# Autodesk Inventor assembly: Сборка3
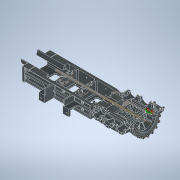
[picture p0: Inventor's stored thumbnail of the model, 180x180]
Saved by Autodesk Inventor 2021 (Build 250183000, 183)
## iProperties
Created: 2020-11-22
Part Number: Сборка3
Document SubType Name: Assembly
Designer: Тимоха
Author: Тимоха
## Documents named in this file (55)
- C:\Users\Тимоха\Desktop\КР Компрессор\compressor\Сборка3.iam
- C:\Users\Тимоха\Desktop\КР Компрессор\compressor\Верхняя часть поршня.ipt
- C:\Users\Тимоха\Desktop\КР Компрессор\compressor\Втулка.ipt
- C:\Users\Тимоха\Desktop\КР Компрессор\compressor\Гайка шток-поршень.ipt
- C:\Users\Тимоха\Desktop\КР Компрессор\compressor\Дроссельное кольцо.ipt
- C:\Users\Тимоха\Desktop\КР Компрессор\compressor\Клапан1.iam
- C:\Users\Тимоха\Desktop\КР Компрессор\compressor\Кольцо поршень-шток верх.ipt
- C:\Users\Тимоха\Desktop\КР Компрессор\compressor\Кольцо поршень-шток низ.ipt
- C:\Users\Тимоха\Desktop\КР Компрессор\compressor\Кольцо поршня.ipt
- C:\Users\Тимоха\Desktop\КР Компрессор\compressor\Кольцо сальника.ipt
- C:\Users\Тимоха\Desktop\КР Компрессор\compressor\Корпус дросселя.ipt
- C:\Users\Тимоха\Desktop\КР Компрессор\compressor\Корпус сальника.ipt
- C:\Users\Тимоха\Desktop\КР Компрессор\compressor\Крышка сальников.ipt
- C:\Users\Тимоха\Desktop\КР Компрессор\compressor\Крышка стакана.ipt
- C:\Users\Тимоха\Desktop\КР Компрессор\compressor\Крышка цилиндра 1.ipt
- C:\Users\Тимоха\Desktop\КР Компрессор\compressor\Крышка цилиндра 2.ipt
- C:\Users\Тимоха\Desktop\КР Компрессор\compressor\Нижняя часть поршня.ipt
- C:\Users\Тимоха\Desktop\КР Компрессор\compressor\Опорное кольцо.ipt
- C:\Users\Тимоха\Desktop\КР Компрессор\compressor\Прокладка клапана.ipt
- C:\Users\Тимоха\Desktop\КР Компрессор\compressor\Пружина дросселя.ipt
- C:\Users\Тимоха\Desktop\КР Компрессор\compressor\Пружина сальника.ipt
- C:\Users\Тимоха\Desktop\КР Компрессор\compressor\Стакан1.ipt
- C:\Users\Тимоха\Desktop\КР Компрессор\compressor\Цилиндр2.ipt
- C:\Users\Тимоха\Desktop\КР Компрессор\compressor\Шток.ipt
- C:\Users\Тимоха\Desktop\КР Компрессор\compressor\Прокладка сальников.ipt
- C:\Users\Тимоха\Documents\Inventor\Content Center Files\R2021\ru-RU\Stud GOST 22034-76\Шпилька M20-6g×50 ГОСТ 22034-76.ipt
- C:\Users\Тимоха\Documents\Inventor\Content Center Files\R2021\ru-RU\GOST 10450-78\Шайба 21 ГОСТ 10450-78.ipt
- C:\Users\Тимоха\Documents\Inventor\Content Center Files\R2021\ru-RU\GOST 15521-70\Гайка M20-6H ГОСТ 15521-70.ipt
- C:\Users\Тимоха\Documents\Inventor\Content Center Files\R2021\ru-RU\GOST 11371-78  A\Шайба 24 ГОСТ 11371-78.ipt
- C:\Users\Тимоха\Documents\Inventor\Content Center Files\R2021\ru-RU\Stud GOST 22038-76\Шпилька M24-6g×70 ГОСТ 22038-76.ipt
- C:\Users\Тимоха\Documents\Inventor\Content Center Files\R2021\ru-RU\Nut GOST 15524-70\Гайка M24-6H ГОСТ 15524-70.ipt
- C:\Users\Тимоха\Documents\Inventor\Content Center Files\R2021\ru-RU\Bolt GOST R 50274-92\Болт M8-6g×20-F ГОСТ Р 50274-92.ipt
- C:\Users\Тимоха\Desktop\КР Компрессор\compressor\Деталь5.ipt
- C:\Users\Тимоха\Desktop\КР Компрессор\compressor\Деталь6.ipt
- C:\Users\Тимоха\Desktop\КР Компрессор\compressor\Прокладка воды зад.ipt
- C:\Users\Тимоха\Desktop\КР Компрессор\compressor\Крышка воды зад.ipt
- C:\Users\Тимоха\Documents\Inventor\Content Center Files\R2021\ru-RU\GOST 15521-70\Гайка M10-6H ГОСТ 15521-70.ipt
- C:\Users\Тимоха\Documents\Inventor\Content Center Files\R2021\ru-RU\Stud GOST 22034-76\Шпилька M10-6g×45 ГОСТ 22034-76.ipt
- C:\Users\Тимоха\Documents\Inventor\Content Center Files\R2021\ru-RU\Washer GOST 9065-75\Шайба 12 ГОСТ 9065-75.ipt
- C:\Users\Тимоха\Desktop\КР Компрессор\compressor\Фонарь.ipt
- C:\Users\Тимоха\Documents\Inventor\Content Center Files\R2021\ru-RU\Stud GOST 22038-76\Шпилька M20-6g×80 ГОСТ 22038-76.ipt
- C:\Users\Тимоха\Documents\Inventor\Content Center Files\R2021\ru-RU\GOST 6402-70\Шайба  22 L ГОСТ 6402-70.ipt
- C:\Users\Тимоха\Documents\Inventor\Content Center Files\R2021\ru-RU\Nut GOST ISO 8673-2014\Копия Копия гайки M20x1,5-6H ГОСТ 5915-70.ipt
- C:\Users\Тимоха\Desktop\КР Компрессор\compressor\Корпус сальника перегородка 1.ipt
- C:\Users\Тимоха\Desktop\КР Компрессор\compressor\Крышка перегородки11.ipt
- C:\Users\Тимоха\Desktop\КР Компрессор\compressor\Крышка перегородки12.ipt
- C:\Users\Тимоха\Desktop\КР Компрессор\compressor\Придав перегородки1.ipt
- C:\Users\Тимоха\Desktop\КР Компрессор\compressor\Корпус маслосъемника.ipt
- C:\Users\Тимоха\Desktop\КР Компрессор\compressor\Крышка перегородки21.ipt
- C:\Users\Тимоха\Desktop\КР Компрессор\compressor\Крышка перегородки22.ipt
- C:\Users\Тимоха\Desktop\КР Компрессор\compressor\Маслосъемная пружина.ipt
- C:\Users\Тимоха\Desktop\КР Компрессор\compressor\Маслосъемное кольцо.ipt
- C:\Users\Тимоха\Documents\Inventor\Content Center Files\R2021\ru-RU\GOST 11738-84\Винт M10-6gx20 ГОСТ 11738-84.ipt
- C:\Users\Тимоха\Documents\Inventor\Content Center Files\R2021\ru-RU\GOST 11371-78  A\Шайба 12 ГОСТ 11371-78.ipt
- C:\Users\Тимоха\Documents\Inventor\Content Center Files\R2021\ru-RU\GOST 11738-84\Винт M10-6gx25 ГОСТ 11738-84.ipt
## Components (444 placed, 54 different names)
1. Верхняя часть поршня:1 — С поворотом:1, С поворотом:2, Жесткий:3, Жесткий:6
2. Втулка:1 — Жесткий:9, Жесткий:12, Жесткий:14
3. Дроссельное кольцо:1 — Жесткий:21, Жесткий:22
4. Клапан1:1 [sub-assembly] — Жесткий:11, С поворотом:4
5. Кольцо поршень-шток низ:1 — Жесткий:5
6. Кольцо поршня:1 — С поворотом:2
7. Корпус дросселя:1 — Жесткий:22, С поворотом:6, С поворотом:7
8. Крышка сальников:1 — Жесткий:72, Жесткий:73, Жесткий:143
9. Крышка стакана:1 — С поворотом:5
10. Крышка цилиндра 1:1 — Жесткий:12, С поворотом:9
11. Крышка цилиндра 2:1 — Жесткий:13, С поворотом:6, Жесткий:79, Жесткий:142, Жесткий:145, С поворотом:16
12. Нижняя часть поршня:1 — С поворотом:1, Жесткий:1, Жесткий:2, Жесткий:4, Жесткий:5
13. Опорное кольцо:1 — Жесткий:4
14. Прокладка клапана:1 — Жесткий:10, Жесткий:11
15. Пружина дросселя:1 — Жесткий:21
16. Стакан1:1 — С поворотом:4, С поворотом:5
17. Цилиндр2:1 — Жесткий:9, Жесткий:10, Жесткий:13, Жесткий:74, Жесткий:76, Жесткий:80, Заподлицо:1, Заподлицо:2, Заподлицо:5, Заподлицо:6
18. Кольцо поршня:2 — Жесткий:1, Жесткий:14
19. Кольцо поршня:3 — Жесткий:2
20. Опорное кольцо:2 — Жесткий:3
21. Гайка шток-поршень:1 — Жесткий:7, Жесткий:8
22. Кольцо поршень-шток верх:1 — Жесткий:6, Жесткий:7
23. Шток:1 — Жесткий:8
24. Прокладка сальников:1 — Жесткий:29, С поворотом:7
25. Кольцо сальника:4
26. Корпус сальника:2 — Жесткий:29, Жесткий:65
27. Пружина сальника:4
28. Кольцо сальника:5
29. Пружина сальника:5
30. Кольцо сальника:6
31. Пружина сальника:6
32. Прокладка сальников:2
33. Кольцо сальника:7
34. Корпус сальника:3 — Жесткий:69, Жесткий:73
35. Пружина сальника:7
36. Кольцо сальника:8
37. Пружина сальника:8
38. Кольцо сальника:9
39. Пружина сальника:9
40. Прокладка сальников:3
41. Кольцо сальника:10
42. Корпус сальника:4 — Жесткий:66, Жесткий:67
43. Пружина сальника:10
44. Кольцо сальника:11
45. Пружина сальника:11
46. Кольцо сальника:12
47. Пружина сальника:12
48. Прокладка сальников:4 — Жесткий:67
49. Кольцо сальника:13
50. Корпус сальника:5 — Жесткий:68
51. Пружина сальника:13
52. Кольцо сальника:14
53. Пружина сальника:14
54. Кольцо сальника:15
55. Пружина сальника:15
56. Прокладка сальников:5
57. Кольцо сальника:16
58. Корпус сальника:6 — Жесткий:68, Жесткий:69
59. Пружина сальника:16
60. Кольцо сальника:17
61. Пружина сальника:17
62. Кольцо сальника:18
63. Пружина сальника:18
64. Прокладка сальников:6
65. Кольцо сальника:19
66. Корпус сальника:7 — Жесткий:65, Жесткий:66
67. Пружина сальника:19
68. Кольцо сальника:20
69. Пружина сальника:20
70. Кольцо сальника:21
71. Пружина сальника:21
72. Кольцо сальника:22 — Жесткий:70, Жесткий:140
73. Кольцо сальника:23 — Жесткий:70, Жесткий:71, Жесткий:139
74. Кольцо сальника:24 — Жесткий:71, Жесткий:72, Жесткий:141
75. Болт ГОСТ Р 50274-92 M8-6g×20-F:2 — Жесткий:82
76. Болт ГОСТ Р 50274-92 M8-6g×20-F:3 — Жесткий:81
77. Деталь5:1 — Заподлицо:1, Заподлицо:2, Заподлицо:3, Заподлицо:4
78. Деталь6:1 — Заподлицо:3, Заподлицо:4, Жесткий:81, Жесткий:82, С поворотом:10, С поворотом:11, С поворотом:12, С поворотом:13, С поворотом:14, Жесткий:83, Жесткий:84, Жесткий:85, Жесткий:86, Жесткий:87, Жесткий:88, Жесткий:89, Жесткий:90, Жесткий:91, Жесткий:92, Жесткий:93, Жесткий:94, Жесткий:95, Жесткий:96, Жесткий:97, Жесткий:98, Жесткий:99, Жесткий:100, Жесткий:101, Жесткий:102, Жесткий:103, Жесткий:104, Жесткий:105, Жесткий:106, Жесткий:107
79. Прокладка воды зад:1 — Заподлицо:5, Заподлицо:6, Заподлицо:7, Заподлицо:8
80. Крышка воды зад:1 — Заподлицо:7, Заподлицо:8, С поворотом:15, Жесткий:108, Жесткий:109, Жесткий:110, Жесткий:111, Жесткий:112, Жесткий:113, Жесткий:114, Жесткий:115, Жесткий:116, Жесткий:117, Жесткий:118, Жесткий:119, Жесткий:120, Жесткий:121, Жесткий:122, Жесткий:123, Жесткий:124, Жесткий:125, Жесткий:126, Жесткий:127, Жесткий:128, Жесткий:129, Жесткий:130, Жесткий:131, Жесткий:132, Жесткий:133, Жесткий:134, Жесткий:135, Жесткий:136, Жесткий:137, Жесткий:138
81. Болт ГОСТ Р 50274-92 M8-6g×20-F:33 — С поворотом:14
82. Болт ГОСТ Р 50274-92 M8-6g×20-F:34 — Жесткий:85
83. Болт ГОСТ Р 50274-92 M8-6g×20-F:35 — С поворотом:11
84. Болт ГОСТ Р 50274-92 M8-6g×20-F:36 — С поворотом:10
85. Болт ГОСТ Р 50274-92 M8-6g×20-F:37 — Жесткий:83
86. Болт ГОСТ Р 50274-92 M8-6g×20-F:38 — Жесткий:84
87. Болт ГОСТ Р 50274-92 M8-6g×20-F:39 — С поворотом:12
88. Болт ГОСТ Р 50274-92 M8-6g×20-F:40 — С поворотом:13
89. Болт ГОСТ Р 50274-92 M8-6g×20-F:41 — Жесткий:91
90. Болт ГОСТ Р 50274-92 M8-6g×20-F:42 — Жесткий:90
91. Болт ГОСТ Р 50274-92 M8-6g×20-F:43 — Жесткий:87
92. Болт ГОСТ Р 50274-92 M8-6g×20-F:44 — Жесткий:86
93. Болт ГОСТ Р 50274-92 M8-6g×20-F:45 — Жесткий:89
94. Болт ГОСТ Р 50274-92 M8-6g×20-F:46 — Жесткий:93
95. Болт ГОСТ Р 50274-92 M8-6g×20-F:47 — Жесткий:88
96. Болт ГОСТ Р 50274-92 M8-6g×20-F:48 — Жесткий:92
97. Болт ГОСТ Р 50274-92 M8-6g×20-F:49 — Жесткий:99
98. Болт ГОСТ Р 50274-92 M8-6g×20-F:50 — Жесткий:98
99. Болт ГОСТ Р 50274-92 M8-6g×20-F:51 — Жесткий:97
100. Болт ГОСТ Р 50274-92 M8-6g×20-F:52 — Жесткий:94
101. Болт ГОСТ Р 50274-92 M8-6g×20-F:53 — Жесткий:95
102. Болт ГОСТ Р 50274-92 M8-6g×20-F:54 — Жесткий:102
103. Болт ГОСТ Р 50274-92 M8-6g×20-F:55 — Жесткий:100
104. Болт ГОСТ Р 50274-92 M8-6g×20-F:56 — Жесткий:101
105. Болт ГОСТ Р 50274-92 M8-6g×20-F:58 — Жесткий:106
106. Болт ГОСТ Р 50274-92 M8-6g×20-F:59 — Жесткий:104
107. Болт ГОСТ Р 50274-92 M8-6g×20-F:60 — Жесткий:96
108. Болт ГОСТ Р 50274-92 M8-6g×20-F:61 — Жесткий:107
109. Болт ГОСТ Р 50274-92 M8-6g×20-F:63 — Жесткий:103
110. Болт ГОСТ Р 50274-92 M8-6g×20-F:64 — Жесткий:105
111. Болт ГОСТ Р 50274-92 M8-6g×20-F:68 — С поворотом:15
112. Болт ГОСТ Р 50274-92 M8-6g×20-F:97 — Жесткий:108
113. Болт ГОСТ Р 50274-92 M8-6g×20-F:98 — Жесткий:110
114. Болт ГОСТ Р 50274-92 M8-6g×20-F:99 — Жесткий:109
115. Болт ГОСТ Р 50274-92 M8-6g×20-F:100 — Жесткий:111
116. Болт ГОСТ Р 50274-92 M8-6g×20-F:101 — Жесткий:113
117. Болт ГОСТ Р 50274-92 M8-6g×20-F:102 — Жесткий:112
118. Болт ГОСТ Р 50274-92 M8-6g×20-F:103 — Жесткий:114
119. Болт ГОСТ Р 50274-92 M8-6g×20-F:104 — Жесткий:115
120. Болт ГОСТ Р 50274-92 M8-6g×20-F:105 — Жесткий:116
121. Болт ГОСТ Р 50274-92 M8-6g×20-F:106 — Жесткий:118
122. Болт ГОСТ Р 50274-92 M8-6g×20-F:107 — Жесткий:130
123. Болт ГОСТ Р 50274-92 M8-6g×20-F:108 — Жесткий:134
124. Болт ГОСТ Р 50274-92 M8-6g×20-F:109 — Жесткий:133
125. Болт ГОСТ Р 50274-92 M8-6g×20-F:110 — Жесткий:131
126. Болт ГОСТ Р 50274-92 M8-6g×20-F:111 — Жесткий:135
127. Болт ГОСТ Р 50274-92 M8-6g×20-F:112 — Жесткий:132
128. Болт ГОСТ Р 50274-92 M8-6g×20-F:117 — Жесткий:117
129. Болт ГОСТ Р 50274-92 M8-6g×20-F:118 — Жесткий:119
130. Болт ГОСТ Р 50274-92 M8-6g×20-F:119 — Жесткий:120
131. Болт ГОСТ Р 50274-92 M8-6g×20-F:120 — Жесткий:121
132. Болт ГОСТ Р 50274-92 M8-6g×20-F:121 — Жесткий:122
133. Болт ГОСТ Р 50274-92 M8-6g×20-F:122 — Жесткий:123
134. Болт ГОСТ Р 50274-92 M8-6g×20-F:123 — Жесткий:124
135. Болт ГОСТ Р 50274-92 M8-6g×20-F:124 — Жесткий:125
136. Болт ГОСТ Р 50274-92 M8-6g×20-F:125 — Жесткий:126
137. Болт ГОСТ Р 50274-92 M8-6g×20-F:126 — Жесткий:127
138. Болт ГОСТ Р 50274-92 M8-6g×20-F:130 — Жесткий:129
139. Болт ГОСТ Р 50274-92 M8-6g×20-F:137 — Жесткий:128
140. Болт ГОСТ Р 50274-92 M8-6g×20-F:138 — Жесткий:137
141. Болт ГОСТ Р 50274-92 M8-6g×20-F:139 — Жесткий:136
142. Болт ГОСТ Р 50274-92 M8-6g×20-F:140 — Жесткий:138
143. Пружина сальника:22 — Жесткий:141
144. Пружина сальника:23 — Жесткий:140
145. Пружина сальника:24 — Жесткий:139
146. Фонарь:1 — Жесткий:145, Жесткий:146, Жесткий:160, Жесткий:168
147. Кольцо сальника:25 — Жесткий:148, Жесткий:152
148. Корпус сальника перегородка 1:1 — Жесткий:158, Жесткий:159, Жесткий:161, Жесткий:162
149. Крышка перегородки11:1 — Жесткий:160, Жесткий:161, Жесткий:163
150. Крышка перегородки12:1 — Жесткий:162, Жесткий:188
151. Придав перегородки1:1 — Жесткий:163, Жесткий:184
152. Пружина сальника:25 — Жесткий:148
153. Кольцо сальника:26 — Жесткий:151, Жесткий:158
154. Пружина сальника:26
155. Кольцо сальника:27 — Жесткий:151, Жесткий:152
156. Пружина сальника:27
157. Кольцо сальника:28 — Жесткий:159
158. Пружина сальника:28
159. Кольцо сальника:29
160. Пружина сальника:29
161. Кольцо сальника:30
162. Пружина сальника:30
163. Корпус маслосъемника:1 — Жесткий:167, Жесткий:175
164. Крышка перегородки21:1 — Жесткий:168, Жесткий:174, Жесткий:175, Жесткий:176, Жесткий:179
165. Крышка перегородки22:1 — Жесткий:176, Жесткий:185
166. Маслосъемное кольцо:1 — Жесткий:166, Жесткий:177
167. Придав перегородки1:2 — Жесткий:179, Жесткий:180
168. Маслосъемное кольцо:2 — Жесткий:166, Жесткий:167, Жесткий:178
169. Кольцо сальника:31 — Жесткий:174
170. Пружина сальника:31
171. Кольцо сальника:32
172. Пружина сальника:32
173. Кольцо сальника:33
174. Пружина сальника:33
175. Маслосъемная пружина:3 — Жесткий:177
176. Маслосъемная пружина:4 — Жесткий:178
177. Гайка ГОСТ 15524-70 M24:1 — Жесткий:77
178. Шайба  ГОСТ 11371-78 25:1 — Жесткий:77, С поворотом:9
179. Шпилька ГОСТ 22038-76 M24-6g×70:1 — Жесткий:76
180. Гайка ГОСТ 15524-70 M24:2
181. Шайба  ГОСТ 11371-78 25:2
182. Шпилька ГОСТ 22038-76 M24-6g×70:2
183. Гайка ГОСТ 15524-70 M24:3
184. Шайба  ГОСТ 11371-78 25:3
185. Шпилька ГОСТ 22038-76 M24-6g×70:3
186. Гайка ГОСТ 15524-70 M24:4
187. Шайба  ГОСТ 11371-78 25:4
188. Шпилька ГОСТ 22038-76 M24-6g×70:4
189. Гайка ГОСТ 15524-70 M24:5
190. Шайба  ГОСТ 11371-78 25:5
191. Шпилька ГОСТ 22038-76 M24-6g×70:5
192. Гайка ГОСТ 15524-70 M24:6
193. Шайба  ГОСТ 11371-78 25:6
194. Шпилька ГОСТ 22038-76 M24-6g×70:6
195. Гайка ГОСТ 15524-70 M24:7
196. Шайба  ГОСТ 11371-78 25:7
197. Шпилька ГОСТ 22038-76 M24-6g×70:7
198. Гайка ГОСТ 15524-70 M24:8
199. Шайба  ГОСТ 11371-78 25:8
200. Шпилька ГОСТ 22038-76 M24-6g×70:8
201. Гайка ГОСТ 15524-70 M24:9
202. Шайба  ГОСТ 11371-78 25:9
203. Шпилька ГОСТ 22038-76 M24-6g×70:9
204. Гайка ГОСТ 15524-70 M24:10
205. Шайба  ГОСТ 11371-78 25:10
206. Шпилька ГОСТ 22038-76 M24-6g×70:10
207. Гайка ГОСТ 15524-70 M24:11
208. Шайба  ГОСТ 11371-78 25:11
209. Шпилька ГОСТ 22038-76 M24-6g×70:11
210. Гайка ГОСТ 15524-70 M24:12
211. Шайба  ГОСТ 11371-78 25:12
212. Шпилька ГОСТ 22038-76 M24-6g×70:12
213. Гайка ГОСТ 15524-70 M24:13
214. Шайба  ГОСТ 11371-78 25:13
215. Шпилька ГОСТ 22038-76 M24-6g×70:13
216. Гайка ГОСТ 15524-70 M24:14
217. Шайба  ГОСТ 11371-78 25:14
218. Шпилька ГОСТ 22038-76 M24-6g×70:14
219. Гайка ГОСТ 15524-70 M24:15
220. Шайба  ГОСТ 11371-78 25:15
221. Шпилька ГОСТ 22038-76 M24-6g×70:15
222. Гайка ГОСТ 15524-70 M24:16
223. Шайба  ГОСТ 11371-78 25:16
224. Шпилька ГОСТ 22038-76 M24-6g×70:16
225. Шпилька ГОСТ 22038-76 M24-6g×70:17 — Жесткий:80
226. Гайка ГОСТ 15524-70 M24:17
227. Шайба  ГОСТ 11371-78 25:17 — Жесткий:79
228. Шпилька ГОСТ 22038-76 M24-6g×70:18
229. Гайка ГОСТ 15524-70 M24:18
230. Шайба  ГОСТ 11371-78 25:18
231. Шпилька ГОСТ 22038-76 M24-6g×70:19
232. Гайка ГОСТ 15524-70 M24:19
233. Шайба  ГОСТ 11371-78 25:19
234. Шпилька ГОСТ 22038-76 M24-6g×70:20
235. Гайка ГОСТ 15524-70 M24:20
236. Шайба  ГОСТ 11371-78 25:20
237. Шпилька ГОСТ 22038-76 M24-6g×70:21
238. Гайка ГОСТ 15524-70 M24:21
239. Шайба  ГОСТ 11371-78 25:21
240. Шпилька ГОСТ 22038-76 M24-6g×70:22
241. Гайка ГОСТ 15524-70 M24:22
242. Шайба  ГОСТ 11371-78 25:22
243. Шпилька ГОСТ 22038-76 M24-6g×70:23
244. Гайка ГОСТ 15524-70 M24:23
245. Шайба  ГОСТ 11371-78 25:23
246. Шпилька ГОСТ 22038-76 M24-6g×70:24
247. Гайка ГОСТ 15524-70 M24:24
248. Шайба  ГОСТ 11371-78 25:24
249. Шпилька ГОСТ 22038-76 M24-6g×70:25
250. Гайка ГОСТ 15524-70 M24:25
251. Шайба  ГОСТ 11371-78 25:25
252. Шпилька ГОСТ 22038-76 M24-6g×70:26
253. Гайка ГОСТ 15524-70 M24:26
254. Шайба  ГОСТ 11371-78 25:26
255. Шпилька ГОСТ 22038-76 M24-6g×70:27
256. Гайка ГОСТ 15524-70 M24:27
257. Шайба  ГОСТ 11371-78 25:27
258. Шпилька ГОСТ 22038-76 M24-6g×70:28
259. Гайка ГОСТ 15524-70 M24:28
260. Шайба  ГОСТ 11371-78 25:28
261. Шпилька ГОСТ 22038-76 M24-6g×70:29
262. Гайка ГОСТ 15524-70 M24:29
263. Шайба  ГОСТ 11371-78 25:29
264. Шпилька ГОСТ 22038-76 M24-6g×70:30
265. Гайка ГОСТ 15524-70 M24:30
266. Шайба  ГОСТ 11371-78 25:30
267. Шпилька ГОСТ 22038-76 M24-6g×70:31
268. Гайка ГОСТ 15524-70 M24:31
269. Шайба  ГОСТ 11371-78 25:31
270. Шпилька ГОСТ 22038-76 M24-6g×70:32
271. Гайка ГОСТ 15524-70 M24:32
272. Шайба  ГОСТ 11371-78 25:32
273. Шпилька ГОСТ 22034-76 M10-6g×45:1 — Жесткий:142
274. Гайка ГОСТ 15521-70 M10:1 — Жесткий:144
275. Шайба ГОСТ 9065-75 12:1 — Жесткий:143, Жесткий:144
276. Шпилька ГОСТ 22034-76 M10-6g×45:2
277. Гайка ГОСТ 15521-70 M10:2
278. Шайба ГОСТ 9065-75 12:2
279. Шпилька ГОСТ 22034-76 M10-6g×45:3
280. Гайка ГОСТ 15521-70 M10:3
281. Шайба ГОСТ 9065-75 12:3
282. Шпилька ГОСТ 22034-76 M10-6g×45:4
283. Гайка ГОСТ 15521-70 M10:4
284. Шайба ГОСТ 9065-75 12:4
285. Шпилька ГОСТ 22034-76 M10-6g×45:5
286. Гайка ГОСТ 15521-70 M10:5
287. Шайба ГОСТ 9065-75 12:5
288. Шпилька ГОСТ 22034-76 M10-6g×45:6
289. Гайка ГОСТ 15521-70 M10:6
290. Шайба ГОСТ 9065-75 12:6
291. Шпилька ГОСТ 22034-76 M10-6g×45:7
292. Гайка ГОСТ 15521-70 M10:7
293. Шайба ГОСТ 9065-75 12:7
294. Шпилька ГОСТ 22034-76 M10-6g×45:8
295. Гайка ГОСТ 15521-70 M10:8
296. Шайба ГОСТ 9065-75 12:8
297. Шпилька ГОСТ 22034-76 M10-6g×45:9
298. Гайка ГОСТ 15521-70 M10:9
299. Шайба ГОСТ 9065-75 12:9
300. Шпилька ГОСТ 22034-76 M10-6g×45:10
301. Гайка ГОСТ 15521-70 M10:10
302. Шайба ГОСТ 9065-75 12:10
303. Шпилька ГОСТ 22038-76 M20-6g×80:1 — С поворотом:16
304. Гайка ГОСТ ISO 8673-2014 M20x1,5:1 — Жесткий:147
305. Шайба ГОСТ 6402-70 22 L:1 — Жесткий:146, Жесткий:147
306. Шпилька ГОСТ 22038-76 M20-6g×80:2
307. Гайка ГОСТ ISO 8673-2014 M20x1,5:2
308. Шайба ГОСТ 6402-70 22 L:2
309. Шпилька ГОСТ 22038-76 M20-6g×80:3
310. Гайка ГОСТ ISO 8673-2014 M20x1,5:3
311. Шайба ГОСТ 6402-70 22 L:3
312. Шпилька ГОСТ 22038-76 M20-6g×80:4
313. Гайка ГОСТ ISO 8673-2014 M20x1,5:4
314. Шайба ГОСТ 6402-70 22 L:4
315. Шпилька ГОСТ 22038-76 M20-6g×80:5
316. Гайка ГОСТ ISO 8673-2014 M20x1,5:5
317. Шайба ГОСТ 6402-70 22 L:5
318. Шпилька ГОСТ 22038-76 M20-6g×80:6
319. Гайка ГОСТ ISO 8673-2014 M20x1,5:6
320. Шайба ГОСТ 6402-70 22 L:6
321. Шпилька ГОСТ 22038-76 M20-6g×80:7
322. Гайка ГОСТ ISO 8673-2014 M20x1,5:7
323. Шайба ГОСТ 6402-70 22 L:7
324. Шпилька ГОСТ 22038-76 M20-6g×80:8
325. Гайка ГОСТ ISO 8673-2014 M20x1,5:8
326. Шайба ГОСТ 6402-70 22 L:8
327. Шпилька ГОСТ 22038-76 M20-6g×80:9
328. Гайка ГОСТ ISO 8673-2014 M20x1,5:9
329. Шайба ГОСТ 6402-70 22 L:9
330. Шпилька ГОСТ 22038-76 M20-6g×80:10
331. Гайка ГОСТ ISO 8673-2014 M20x1,5:10
332. Шайба ГОСТ 6402-70 22 L:10
333. Шпилька ГОСТ 22038-76 M20-6g×80:11
334. Гайка ГОСТ ISO 8673-2014 M20x1,5:11
335. Шайба ГОСТ 6402-70 22 L:11
336. Шпилька ГОСТ 22038-76 M20-6g×80:12
337. Гайка ГОСТ ISO 8673-2014 M20x1,5:12
338. Шайба ГОСТ 6402-70 22 L:12
339. Шпилька ГОСТ 22038-76 M20-6g×80:13
340. Гайка ГОСТ ISO 8673-2014 M20x1,5:13
341. Шайба ГОСТ 6402-70 22 L:13
342. Шпилька ГОСТ 22038-76 M20-6g×80:14
343. Гайка ГОСТ ISO 8673-2014 M20x1,5:14
344. Шайба ГОСТ 6402-70 22 L:14
345. Шпилька ГОСТ 22038-76 M20-6g×80:15
346. Гайка ГОСТ ISO 8673-2014 M20x1,5:15
347. Шайба ГОСТ 6402-70 22 L:15
348. Шпилька ГОСТ 22038-76 M20-6g×80:16
349. Гайка ГОСТ ISO 8673-2014 M20x1,5:16
350. Шайба ГОСТ 6402-70 22 L:16
351. Гайка ГОСТ 15521-70 M20:1 — Жесткий:75
352. Шпилька ГОСТ 22034-76 M20-6g×50:1 — Жесткий:74, Жесткий:75
353. Шайба ГОСТ 10450-78 21:1
354. Гайка ГОСТ 15521-70 M20:2
355. Шпилька ГОСТ 22034-76 M20-6g×50:2
356. Шайба ГОСТ 10450-78 21:2
357. Гайка ГОСТ 15521-70 M20:3
358. Шпилька ГОСТ 22034-76 M20-6g×50:3
359. Шайба ГОСТ 10450-78 21:3
360. Гайка ГОСТ 15521-70 M20:4
361. Шпилька ГОСТ 22034-76 M20-6g×50:4
362. Шайба ГОСТ 10450-78 21:4
363. Гайка ГОСТ 15521-70 M20:5
364. Шпилька ГОСТ 22034-76 M20-6g×50:5
365. Шайба ГОСТ 10450-78 21:5
366. Гайка ГОСТ 15521-70 M20:6
367. Шпилька ГОСТ 22034-76 M20-6g×50:6
368. Шайба ГОСТ 10450-78 21:6
369. Гайка ГОСТ 15521-70 M20:7
370. Шпилька ГОСТ 22034-76 M20-6g×50:7
371. Шайба ГОСТ 10450-78 21:7
372. Гайка ГОСТ 15521-70 M20:8
373. Шпилька ГОСТ 22034-76 M20-6g×50:8
374. Шайба ГОСТ 10450-78 21:8
375. Гайка ГОСТ 15521-70 M20:9
376. Шпилька ГОСТ 22034-76 M20-6g×50:9
377. Шайба ГОСТ 10450-78 21:9
378. Гайка ГОСТ 15521-70 M20:10
379. Шпилька ГОСТ 22034-76 M20-6g×50:10
380. Шайба ГОСТ 10450-78 21:10
381. Винт ГОСТ 11738-84 M 10x20:1 — Жесткий:181
382. Шайба  ГОСТ 11371-78 13:1 — Жесткий:180, Жесткий:181
383. Винт ГОСТ 11738-84 M 10x20:4
384. Шайба  ГОСТ 11371-78 13:4
385. Винт ГОСТ 11738-84 M 10x20:5
386. Шайба  ГОСТ 11371-78 13:5
387. Винт ГОСТ 11738-84 M 10x20:6
388. Шайба  ГОСТ 11371-78 13:6
389. Винт ГОСТ 11738-84 M 10x20:7
390. Шайба  ГОСТ 11371-78 13:7
391. Винт ГОСТ 11738-84 M 10x20:8
392. Шайба  ГОСТ 11371-78 13:8
393. Винт ГОСТ 11738-84 M 10x20:9
394. Шайба  ГОСТ 11371-78 13:9
395. Винт ГОСТ 11738-84 M 10x20:10
396. Шайба  ГОСТ 11371-78 13:10
397. Винт ГОСТ 11738-84 M 10x20:3
398. Шайба  ГОСТ 11371-78 13:3 — Жесткий:184
399. Винт ГОСТ 11738-84 M 10x20:11
400. Шайба  ГОСТ 11371-78 13:11
401. Винт ГОСТ 11738-84 M 10x20:12
402. Шайба  ГОСТ 11371-78 13:12
403. Винт ГОСТ 11738-84 M 10x20:13
404. Шайба  ГОСТ 11371-78 13:13
405. Винт ГОСТ 11738-84 M 10x20:14
406. Шайба  ГОСТ 11371-78 13:14
407. Винт ГОСТ 11738-84 M 10x20:15
408. Шайба  ГОСТ 11371-78 13:15
409. Винт ГОСТ 11738-84 M 10x20:16
410. Шайба  ГОСТ 11371-78 13:16
411. Винт ГОСТ 11738-84 M 10x20:17
412. Шайба  ГОСТ 11371-78 13:17
413. Винт ГОСТ 11738-84 M 10x25:2
414. Шайба  ГОСТ 11371-78 13:19 — Жесткий:188
415. Винт ГОСТ 11738-84 M 10x25:3
416. Шайба  ГОСТ 11371-78 13:20
417. Винт ГОСТ 11738-84 M 10x25:4
418. Шайба  ГОСТ 11371-78 13:21
419. Винт ГОСТ 11738-84 M 10x25:5
420. Шайба  ГОСТ 11371-78 13:22
421. Винт ГОСТ 11738-84 M 10x25:6
422. Шайба  ГОСТ 11371-78 13:23
423. Винт ГОСТ 11738-84 M 10x25:7
424. Шайба  ГОСТ 11371-78 13:24
425. Винт ГОСТ 11738-84 M 10x25:8
426. Шайба  ГОСТ 11371-78 13:25
427. Винт ГОСТ 11738-84 M 10x25:9
428. Шайба  ГОСТ 11371-78 13:26
429. Шайба  ГОСТ 11371-78 13:18 — Жесткий:185, Жесткий:186
430. Винт ГОСТ 11738-84 M 10x25:1 — Жесткий:186
431. Шайба  ГОСТ 11371-78 13:27
432. Винт ГОСТ 11738-84 M 10x25:10
433. Шайба  ГОСТ 11371-78 13:28
434. Винт ГОСТ 11738-84 M 10x25:11
435. Шайба  ГОСТ 11371-78 13:29
436. Винт ГОСТ 11738-84 M 10x25:12
437. Шайба  ГОСТ 11371-78 13:30
438. Винт ГОСТ 11738-84 M 10x25:13
439. Шайба  ГОСТ 11371-78 13:31
440. Винт ГОСТ 11738-84 M 10x25:14
441. Шайба  ГОСТ 11371-78 13:32
442. Винт ГОСТ 11738-84 M 10x25:15
443. Шайба  ГОСТ 11371-78 13:33
444. Винт ГОСТ 11738-84 M 10x25:16
## Component patterns: (16 elements, first: Гайка ГОСТ 15524-70 M24:1 + Шайба  ГОСТ 11371-78 25:1 + Шпилька ГОСТ 22038-76 M24-6g×70:1), (16 elements, first: Шпилька ГОСТ 22038-76 M24-6g×70:17 + Гайка ГОСТ 15524-70 M24:17 + Шайба  ГОСТ 11371-78 25:17), (10 elements, first: Шпилька ГОСТ 22034-76 M10-6g×45:1 + Гайка ГОСТ 15521-70 M10:1 + Шайба ГОСТ 9065-75 12:1), (16 elements, first: Шпилька ГОСТ 22038-76 M20-6g×80:1 + Гайка ГОСТ ISO 8673-2014 M20x1,5:1 + Шайба ГОСТ 6402-70 22 L:1), (10 elements, first: Гайка ГОСТ 15521-70 M20:1 + Шпилька ГОСТ 22034-76 M20-6g×50:1 + Шайба ГОСТ 10450-78 21:1), (8 elements, first: Винт ГОСТ 11738-84 M 10x20:1 + Шайба  ГОСТ 11371-78 13:1), (8 elements, first: Винт ГОСТ 11738-84 M 10x20:3 + Шайба  ГОСТ 11371-78 13:3), (8 elements, first: Винт ГОСТ 11738-84 M 10x25:2 + Шайба  ГОСТ 11371-78 13:19), (8 elements, first: Шайба  ГОСТ 11371-78 13:18 + Винт ГОСТ 11738-84 M 10x25:1)
## Relationships (202: WeldJoint 179, RevoluteJoint 15, Flush 8)
- С поворотом:1 [RevoluteJoint]: Верхняя часть поршня:1 ↔ Нижняя часть поршня:1
- С поворотом:2 [RevoluteJoint]: Верхняя часть поршня:1 ↔ Кольцо поршня:1
- Жесткий:1 [WeldJoint]: Нижняя часть поршня:1 ↔ Кольцо поршня:2
- Жесткий:2 [WeldJoint]: Нижняя часть поршня:1 ↔ Кольцо поршня:3
- Жесткий:3 [WeldJoint]: Верхняя часть поршня:1 ↔ Опорное кольцо:2
- Жесткий:4 [WeldJoint]: Нижняя часть поршня:1 ↔ Опорное кольцо:1
- Жесткий:5 [WeldJoint]: Кольцо поршень-шток низ:1 ↔ Нижняя часть поршня:1
- Жесткий:6 [WeldJoint]: Верхняя часть поршня:1 ↔ Кольцо поршень-шток верх:1
- Жесткий:7 [WeldJoint]: Гайка шток-поршень:1 ↔ Кольцо поршень-шток верх:1
- Жесткий:8 [WeldJoint]: Гайка шток-поршень:1 ↔ Шток:1
- Жесткий:9 [WeldJoint]: Втулка:1 ↔ Цилиндр2:1
- Жесткий:10 [WeldJoint]: Прокладка клапана:1 ↔ Цилиндр2:1
- Жесткий:11 [WeldJoint]: Клапан1:1 ↔ Прокладка клапана:1
- С поворотом:4 [RevoluteJoint]: Клапан1:1 ↔ Стакан1:1
- С поворотом:5 [RevoluteJoint]: Крышка стакана:1 ↔ Стакан1:1
- Жесткий:12 [WeldJoint]: Втулка:1 ↔ Крышка цилиндра 1:1
- Жесткий:13 [WeldJoint]: Крышка цилиндра 2:1 ↔ Цилиндр2:1
- Жесткий:14 [WeldJoint]: Втулка:1 ↔ Кольцо поршня:2
- Жесткий:21 [WeldJoint] (2 mm): Дроссельное кольцо:1 ↔ Пружина дросселя:1
- Жесткий:22 [WeldJoint]: Дроссельное кольцо:1 ↔ Корпус дросселя:1
- С поворотом:6 [RevoluteJoint]: Корпус дросселя:1 ↔ Крышка цилиндра 2:1
- [WeldJoint] (-1 mm): Кольцо сальника:4 ↔ Пружина сальника:4
- [WeldJoint] (-1 mm): Кольцо сальника:5 ↔ Пружина сальника:5
- [WeldJoint] (-1 mm): Кольцо сальника:6 ↔ Пружина сальника:6
- [WeldJoint]: Кольцо сальника:5 ↔ Кольцо сальника:6
- [WeldJoint]: Кольцо сальника:4 ↔ Кольцо сальника:5
- [WeldJoint]: Корпус сальника:2 ↔ Кольцо сальника:6
- Жесткий:29 [WeldJoint]: Прокладка сальников:1 ↔ Корпус сальника:2
- [WeldJoint] (-1 mm): Кольцо сальника:7 ↔ Пружина сальника:7
- [WeldJoint] (-1 mm): Кольцо сальника:8 ↔ Пружина сальника:8
- [WeldJoint] (-1 mm): Кольцо сальника:9 ↔ Пружина сальника:9
- [WeldJoint]: Кольцо сальника:8 ↔ Кольцо сальника:9
- [WeldJoint]: Кольцо сальника:7 ↔ Кольцо сальника:8
- [WeldJoint]: Корпус сальника:3 ↔ Кольцо сальника:9
- [WeldJoint]: Прокладка сальников:2 ↔ Корпус сальника:3
- [WeldJoint] (-1 mm): Кольцо сальника:10 ↔ Пружина сальника:10
- [WeldJoint] (-1 mm): Кольцо сальника:11 ↔ Пружина сальника:11
- [WeldJoint] (-1 mm): Кольцо сальника:12 ↔ Пружина сальника:12
- [WeldJoint]: Кольцо сальника:11 ↔ Кольцо сальника:12
- [WeldJoint]: Кольцо сальника:10 ↔ Кольцо сальника:11
- [WeldJoint]: Корпус сальника:4 ↔ Кольцо сальника:12
- [WeldJoint]: Прокладка сальников:3 ↔ Корпус сальника:4
- [WeldJoint] (-1 mm): Кольцо сальника:13 ↔ Пружина сальника:13
- [WeldJoint] (-1 mm): Кольцо сальника:14 ↔ Пружина сальника:14
- [WeldJoint] (-1 mm): Кольцо сальника:15 ↔ Пружина сальника:15
- [WeldJoint]: Кольцо сальника:14 ↔ Кольцо сальника:15
- [WeldJoint]: Кольцо сальника:13 ↔ Кольцо сальника:14
- [WeldJoint]: Корпус сальника:5 ↔ Кольцо сальника:15
- [WeldJoint]: Прокладка сальников:4 ↔ Корпус сальника:5
- [WeldJoint] (-1 mm): Кольцо сальника:16 ↔ Пружина сальника:16
- [WeldJoint] (-1 mm): Кольцо сальника:17 ↔ Пружина сальника:17
- [WeldJoint] (-1 mm): Кольцо сальника:18 ↔ Пружина сальника:18
- [WeldJoint]: Кольцо сальника:17 ↔ Кольцо сальника:18
- [WeldJoint]: Кольцо сальника:16 ↔ Кольцо сальника:17
- [WeldJoint]: Корпус сальника:6 ↔ Кольцо сальника:18
- [WeldJoint]: Прокладка сальников:5 ↔ Корпус сальника:6
- [WeldJoint] (-1 mm): Кольцо сальника:19 ↔ Пружина сальника:19
- [WeldJoint] (-1 mm): Кольцо сальника:20 ↔ Пружина сальника:20
- [WeldJoint] (-1 mm): Кольцо сальника:21 ↔ Пружина сальника:21
- [WeldJoint]: Кольцо сальника:20 ↔ Кольцо сальника:21
- [WeldJoint]: Кольцо сальника:19 ↔ Кольцо сальника:20
- [WeldJoint]: Корпус сальника:7 ↔ Кольцо сальника:21
- [WeldJoint]: Прокладка сальников:6 ↔ Корпус сальника:7
- С поворотом:7 [RevoluteJoint]: Корпус дросселя:1 ↔ Прокладка сальников:1
- Жесткий:65 [WeldJoint]: Корпус сальника:2 ↔ Корпус сальника:7
- Жесткий:66 [WeldJoint]: Корпус сальника:4 ↔ Корпус сальника:7
- Жесткий:67 [WeldJoint]: Корпус сальника:4 ↔ Прокладка сальников:4
- Жесткий:68 [WeldJoint]: Корпус сальника:5 ↔ Корпус сальника:6
- Жесткий:69 [WeldJoint]: Корпус сальника:3 ↔ Корпус сальника:6
- Жесткий:70 [WeldJoint]: Кольцо сальника:22 ↔ Кольцо сальника:23
- Жесткий:71 [WeldJoint]: Кольцо сальника:23 ↔ Кольцо сальника:24
- Жесткий:72 [WeldJoint]: Крышка сальников:1 ↔ Кольцо сальника:24
- Жесткий:73 [WeldJoint]: Крышка сальников:1 ↔ Корпус сальника:3
- [RevoluteJoint]: Гайка ГОСТ 15521-70 M20:1 ↔ Шайба ГОСТ 10450-78 21:1
- Жесткий:74 [WeldJoint] (23.5 mm): Цилиндр2:1 ↔ Шпилька ГОСТ 22034-76 M20-6g×50:1
- Жесткий:75 [WeldJoint] (-2.75 mm): Гайка ГОСТ 15521-70 M20:1 ↔ Шпилька ГОСТ 22034-76 M20-6g×50:1
- Жесткий:76 [WeldJoint]: Цилиндр2:1 ↔ Шпилька ГОСТ 22038-76 M24-6g×70:1
- Жесткий:77 [WeldJoint]: Гайка ГОСТ 15524-70 M24:1 ↔ Шайба  ГОСТ 11371-78 25:1
- С поворотом:9 [RevoluteJoint]: Крышка цилиндра 1:1 ↔ Шайба  ГОСТ 11371-78 25:1
- [WeldJoint]: Гайка ГОСТ 15524-70 M24:17 ↔ Шайба  ГОСТ 11371-78 25:17
- Жесткий:79 [WeldJoint]: Крышка цилиндра 2:1 ↔ Шайба  ГОСТ 11371-78 25:17
- Жесткий:80 [WeldJoint]: Цилиндр2:1 ↔ Шпилька ГОСТ 22038-76 M24-6g×70:17
- Заподлицо:1 [Flush]: Цилиндр2:1 ↔ Деталь5:1
- Заподлицо:2 [Flush]: Цилиндр2:1 ↔ Деталь5:1
- Заподлицо:3 [Flush]: Деталь5:1 ↔ Деталь6:1
- Заподлицо:4 [Flush]: Деталь5:1 ↔ Деталь6:1
- Заподлицо:5 [Flush]: Цилиндр2:1 ↔ Прокладка воды зад:1
- Заподлицо:6 [Flush]: Цилиндр2:1 ↔ Прокладка воды зад:1
- Заподлицо:7 [Flush]: Прокладка воды зад:1 ↔ Крышка воды зад:1
- Заподлицо:8 [Flush]: Прокладка воды зад:1 ↔ Крышка воды зад:1
- Жесткий:81 [WeldJoint]: Болт ГОСТ Р 50274-92 M8-6g×20-F:3 ↔ Деталь6:1
- Жесткий:82 [WeldJoint]: Болт ГОСТ Р 50274-92 M8-6g×20-F:2 ↔ Деталь6:1
- С поворотом:10 [RevoluteJoint]: Деталь6:1 ↔ Болт ГОСТ Р 50274-92 M8-6g×20-F:36
- С поворотом:11 [RevoluteJoint]: Деталь6:1 ↔ Болт ГОСТ Р 50274-92 M8-6g×20-F:35
- С поворотом:12 [RevoluteJoint]: Деталь6:1 ↔ Болт ГОСТ Р 50274-92 M8-6g×20-F:39
- С поворотом:13 [RevoluteJoint]: Деталь6:1 ↔ Болт ГОСТ Р 50274-92 M8-6g×20-F:40
- С поворотом:14 [RevoluteJoint]: Деталь6:1 ↔ Болт ГОСТ Р 50274-92 M8-6g×20-F:33
- Жесткий:83 [WeldJoint]: Деталь6:1 ↔ Болт ГОСТ Р 50274-92 M8-6g×20-F:37
- Жесткий:84 [WeldJoint]: Деталь6:1 ↔ Болт ГОСТ Р 50274-92 M8-6g×20-F:38
- Жесткий:85 [WeldJoint]: Деталь6:1 ↔ Болт ГОСТ Р 50274-92 M8-6g×20-F:34
- Жесткий:86 [WeldJoint]: Деталь6:1 ↔ Болт ГОСТ Р 50274-92 M8-6g×20-F:44
- Жесткий:87 [WeldJoint]: Деталь6:1 ↔ Болт ГОСТ Р 50274-92 M8-6g×20-F:43
- Жесткий:88 [WeldJoint]: Деталь6:1 ↔ Болт ГОСТ Р 50274-92 M8-6g×20-F:47
- Жесткий:89 [WeldJoint]: Деталь6:1 ↔ Болт ГОСТ Р 50274-92 M8-6g×20-F:45
- Жесткий:90 [WeldJoint]: Деталь6:1 ↔ Болт ГОСТ Р 50274-92 M8-6g×20-F:42
- Жесткий:91 [WeldJoint]: Деталь6:1 ↔ Болт ГОСТ Р 50274-92 M8-6g×20-F:41
- Жесткий:92 [WeldJoint]: Деталь6:1 ↔ Болт ГОСТ Р 50274-92 M8-6g×20-F:48
- Жесткий:93 [WeldJoint]: Деталь6:1 ↔ Болт ГОСТ Р 50274-92 M8-6g×20-F:46
- Жесткий:94 [WeldJoint]: Деталь6:1 ↔ Болт ГОСТ Р 50274-92 M8-6g×20-F:52
- Жесткий:95 [WeldJoint]: Деталь6:1 ↔ Болт ГОСТ Р 50274-92 M8-6g×20-F:53
- Жесткий:96 [WeldJoint]: Деталь6:1 ↔ Болт ГОСТ Р 50274-92 M8-6g×20-F:60
- Жесткий:97 [WeldJoint]: Деталь6:1 ↔ Болт ГОСТ Р 50274-92 M8-6g×20-F:51
- Жесткий:98 [WeldJoint]: Деталь6:1 ↔ Болт ГОСТ Р 50274-92 M8-6g×20-F:50
- Жесткий:99 [WeldJoint]: Деталь6:1 ↔ Болт ГОСТ Р 50274-92 M8-6g×20-F:49
- Жесткий:100 [WeldJoint]: Деталь6:1 ↔ Болт ГОСТ Р 50274-92 M8-6g×20-F:55
- Жесткий:101 [WeldJoint]: Деталь6:1 ↔ Болт ГОСТ Р 50274-92 M8-6g×20-F:56
- Жесткий:102 [WeldJoint]: Деталь6:1 ↔ Болт ГОСТ Р 50274-92 M8-6g×20-F:54
- Жесткий:103 [WeldJoint]: Деталь6:1 ↔ Болт ГОСТ Р 50274-92 M8-6g×20-F:63
- Жесткий:104 [WeldJoint]: Деталь6:1 ↔ Болт ГОСТ Р 50274-92 M8-6g×20-F:59
- Жесткий:105 [WeldJoint]: Деталь6:1 ↔ Болт ГОСТ Р 50274-92 M8-6g×20-F:64
- Жесткий:106 [WeldJoint]: Деталь6:1 ↔ Болт ГОСТ Р 50274-92 M8-6g×20-F:58
- Жесткий:107 [WeldJoint]: Деталь6:1 ↔ Болт ГОСТ Р 50274-92 M8-6g×20-F:61
- С поворотом:15 [RevoluteJoint]: Крышка воды зад:1 ↔ Болт ГОСТ Р 50274-92 M8-6g×20-F:68
- Жесткий:108 [WeldJoint]: Крышка воды зад:1 ↔ Болт ГОСТ Р 50274-92 M8-6g×20-F:97
- Жесткий:109 [WeldJoint]: Крышка воды зад:1 ↔ Болт ГОСТ Р 50274-92 M8-6g×20-F:99
- Жесткий:110 [WeldJoint]: Крышка воды зад:1 ↔ Болт ГОСТ Р 50274-92 M8-6g×20-F:98
- Жесткий:111 [WeldJoint]: Крышка воды зад:1 ↔ Болт ГОСТ Р 50274-92 M8-6g×20-F:100
- Жесткий:112 [WeldJoint]: Крышка воды зад:1 ↔ Болт ГОСТ Р 50274-92 M8-6g×20-F:102
- Жесткий:113 [WeldJoint]: Крышка воды зад:1 ↔ Болт ГОСТ Р 50274-92 M8-6g×20-F:101
- Жесткий:114 [WeldJoint]: Крышка воды зад:1 ↔ Болт ГОСТ Р 50274-92 M8-6g×20-F:103
- Жесткий:115 [WeldJoint]: Крышка воды зад:1 ↔ Болт ГОСТ Р 50274-92 M8-6g×20-F:104
- Жесткий:116 [WeldJoint]: Крышка воды зад:1 ↔ Болт ГОСТ Р 50274-92 M8-6g×20-F:105
- Жесткий:117 [WeldJoint]: Крышка воды зад:1 ↔ Болт ГОСТ Р 50274-92 M8-6g×20-F:117
- Жесткий:118 [WeldJoint]: Крышка воды зад:1 ↔ Болт ГОСТ Р 50274-92 M8-6g×20-F:106
- Жесткий:119 [WeldJoint]: Крышка воды зад:1 ↔ Болт ГОСТ Р 50274-92 M8-6g×20-F:118
- Жесткий:120 [WeldJoint]: Крышка воды зад:1 ↔ Болт ГОСТ Р 50274-92 M8-6g×20-F:119
- Жесткий:121 [WeldJoint]: Крышка воды зад:1 ↔ Болт ГОСТ Р 50274-92 M8-6g×20-F:120
- Жесткий:122 [WeldJoint]: Крышка воды зад:1 ↔ Болт ГОСТ Р 50274-92 M8-6g×20-F:121
- Жесткий:123 [WeldJoint]: Крышка воды зад:1 ↔ Болт ГОСТ Р 50274-92 M8-6g×20-F:122
- Жесткий:124 [WeldJoint]: Крышка воды зад:1 ↔ Болт ГОСТ Р 50274-92 M8-6g×20-F:123
- Жесткий:125 [WeldJoint]: Крышка воды зад:1 ↔ Болт ГОСТ Р 50274-92 M8-6g×20-F:124
- Жесткий:126 [WeldJoint]: Крышка воды зад:1 ↔ Болт ГОСТ Р 50274-92 M8-6g×20-F:125
- Жесткий:127 [WeldJoint]: Крышка воды зад:1 ↔ Болт ГОСТ Р 50274-92 M8-6g×20-F:126
- Жесткий:128 [WeldJoint]: Крышка воды зад:1 ↔ Болт ГОСТ Р 50274-92 M8-6g×20-F:137
- Жесткий:129 [WeldJoint]: Крышка воды зад:1 ↔ Болт ГОСТ Р 50274-92 M8-6g×20-F:130
- Жесткий:130 [WeldJoint]: Крышка воды зад:1 ↔ Болт ГОСТ Р 50274-92 M8-6g×20-F:107
- Жесткий:131 [WeldJoint]: Крышка воды зад:1 ↔ Болт ГОСТ Р 50274-92 M8-6g×20-F:110
- Жесткий:132 [WeldJoint]: Крышка воды зад:1 ↔ Болт ГОСТ Р 50274-92 M8-6g×20-F:112
- Жесткий:133 [WeldJoint]: Крышка воды зад:1 ↔ Болт ГОСТ Р 50274-92 M8-6g×20-F:109
- Жесткий:134 [WeldJoint]: Крышка воды зад:1 ↔ Болт ГОСТ Р 50274-92 M8-6g×20-F:108
- Жесткий:135 [WeldJoint]: Крышка воды зад:1 ↔ Болт ГОСТ Р 50274-92 M8-6g×20-F:111
- Жесткий:136 [WeldJoint]: Крышка воды зад:1 ↔ Болт ГОСТ Р 50274-92 M8-6g×20-F:139
- Жесткий:137 [WeldJoint]: Крышка воды зад:1 ↔ Болт ГОСТ Р 50274-92 M8-6g×20-F:138
- Жесткий:138 [WeldJoint]: Крышка воды зад:1 ↔ Болт ГОСТ Р 50274-92 M8-6g×20-F:140
- Жесткий:139 [WeldJoint] (1 mm): Кольцо сальника:23 ↔ Пружина сальника:24
- Жесткий:140 [WeldJoint]: Кольцо сальника:22 ↔ Пружина сальника:23
- Жесткий:141 [WeldJoint]: Кольцо сальника:24 ↔ Пружина сальника:22
- Жесткий:142 [WeldJoint]: Крышка цилиндра 2:1 ↔ Шпилька ГОСТ 22034-76 M10-6g×45:1
- Жесткий:143 [WeldJoint]: Крышка сальников:1 ↔ Шайба ГОСТ 9065-75 12:1
- Жесткий:144 [WeldJoint]: Гайка ГОСТ 15521-70 M10:1 ↔ Шайба ГОСТ 9065-75 12:1
- Жесткий:145 [WeldJoint]: Крышка цилиндра 2:1 ↔ Фонарь:1
- С поворотом:16 [RevoluteJoint]: Крышка цилиндра 2:1 ↔ Шпилька ГОСТ 22038-76 M20-6g×80:1
- Жесткий:146 [WeldJoint]: Фонарь:1 ↔ Шайба ГОСТ 6402-70 22 L:1
- Жесткий:147 [WeldJoint]: Гайка ГОСТ ISO 8673-2014 M20x1,5:1 ↔ Шайба ГОСТ 6402-70 22 L:1
- Жесткий:148 [WeldJoint]: Кольцо сальника:25 ↔ Пружина сальника:25
- [WeldJoint]: Кольцо сальника:26 ↔ Пружина сальника:26
- [WeldJoint]: Кольцо сальника:27 ↔ Пружина сальника:27
- Жесткий:151 [WeldJoint]: Кольцо сальника:26 ↔ Кольцо сальника:27
- Жесткий:152 [WeldJoint]: Кольцо сальника:25 ↔ Кольцо сальника:27
- [WeldJoint]: Кольцо сальника:28 ↔ Пружина сальника:28
- [WeldJoint]: Кольцо сальника:29 ↔ Пружина сальника:29
- [WeldJoint]: Кольцо сальника:30 ↔ Пружина сальника:30
- [WeldJoint]: Кольцо сальника:29 ↔ Кольцо сальника:30
- [WeldJoint]: Кольцо сальника:28 ↔ Кольцо сальника:30
- Жесткий:158 [WeldJoint]: Корпус сальника перегородка 1:1 ↔ Кольцо сальника:26
- Жесткий:159 [WeldJoint]: Корпус сальника перегородка 1:1 ↔ Кольцо сальника:28
- Жесткий:160 [WeldJoint]: Фонарь:1 ↔ Крышка перегородки11:1
- Жесткий:161 [WeldJoint]: Корпус сальника перегородка 1:1 ↔ Крышка перегородки11:1
- Жесткий:162 [WeldJoint]: Корпус сальника перегородка 1:1 ↔ Крышка перегородки12:1
- Жесткий:163 [WeldJoint]: Крышка перегородки11:1 ↔ Придав перегородки1:1
- Жесткий:166 [WeldJoint]: Маслосъемное кольцо:1 ↔ Маслосъемное кольцо:2
- Жесткий:167 [WeldJoint]: Корпус маслосъемника:1 ↔ Маслосъемное кольцо:2
- Жесткий:168 [WeldJoint]: Фонарь:1 ↔ Крышка перегородки21:1
- [WeldJoint]: Кольцо сальника:31 ↔ Пружина сальника:31
- [WeldJoint]: Кольцо сальника:32 ↔ Пружина сальника:32
- [WeldJoint]: Кольцо сальника:33 ↔ Пружина сальника:33
- [WeldJoint]: Кольцо сальника:32 ↔ Кольцо сальника:33
- [WeldJoint]: Кольцо сальника:31 ↔ Кольцо сальника:33
- Жесткий:174 [WeldJoint]: Крышка перегородки21:1 ↔ Кольцо сальника:31
- Жесткий:175 [WeldJoint]: Корпус маслосъемника:1 ↔ Крышка перегородки21:1
- Жесткий:176 [WeldJoint]: Крышка перегородки21:1 ↔ Крышка перегородки22:1
- Жесткий:177 [WeldJoint]: Маслосъемное кольцо:1 ↔ Маслосъемная пружина:3
- Жесткий:178 [WeldJoint] (1 mm): Маслосъемное кольцо:2 ↔ Маслосъемная пружина:4
- Жесткий:179 [WeldJoint]: Крышка перегородки21:1 ↔ Придав перегородки1:2
- Жесткий:180 [WeldJoint]: Придав перегородки1:2 ↔ Шайба  ГОСТ 11371-78 13:1
- Жесткий:181 [WeldJoint]: Винт ГОСТ 11738-84 M 10x20:1 ↔ Шайба  ГОСТ 11371-78 13:1
- [WeldJoint]: Винт ГОСТ 11738-84 M 10x20:3 ↔ Шайба  ГОСТ 11371-78 13:3
- Жесткий:184 [WeldJoint]: Придав перегородки1:1 ↔ Шайба  ГОСТ 11371-78 13:3
- Жесткий:185 [WeldJoint]: Крышка перегородки22:1 ↔ Шайба  ГОСТ 11371-78 13:18
- Жесткий:186 [WeldJoint]: Шайба  ГОСТ 11371-78 13:18 ↔ Винт ГОСТ 11738-84 M 10x25:1
- [WeldJoint]: Винт ГОСТ 11738-84 M 10x25:2 ↔ Шайба  ГОСТ 11371-78 13:19
- Жесткий:188 [WeldJoint]: Крышка перегородки12:1 ↔ Шайба  ГОСТ 11371-78 13:19
## Named parameters: d45_d35 = -1 mm, d46_d36_d35 = -1 mm, d47_d37_d35 = -1 mm, d48_d38 = 0 mm, d49_d39 = 0 mm, d50_d40 = 0 mm, d52_d51 = 0 mm, d53_d45_d35 = -1 mm, d54_d46_d36_d35 = -1 mm, d55_d47_d37_d35 = -1 mm, d56_d48_d38 = 0 mm, d57_d49_d39 = 0 mm, d58_d50_d40 = 0 mm, d59_d51 = 0 mm, d60_d45_d35 = -1 mm, d61_d46_d36_d35 = -1 mm, d62_d47_d37_d35 = -1 mm, d63_d48_d38 = 0 mm, d64_d49_d39 = 0 mm, d65_d50_d40 = 0 mm, d66_d51 = 0 mm, d67_d45_d35 = -1 mm, d68_d46_d36_d35 = -1 mm, d69_d47_d37_d35 = -1 mm, d70_d48_d38 = 0 mm, d71_d49_d39 = 0 mm, d72_d50_d40 = 0 mm, d73_d51 = 0 mm, d74_d45_d35 = -1 mm, d75_d46_d36_d35 = -1 mm, d76_d47_d37_d35 = -1 mm, d77_d48_d38 = 0 mm, d78_d49_d39 = 0 mm, d79_d50_d40 = 0 mm, d80_d51 = 0 mm, d81_d45_d35 = -1 mm, d82_d46_d36_d35 = -1 mm, d83_d47_d37_d35 = -1 mm, d84_d48_d38 = 0 mm, d85_d49_d39 = 0 mm, d86_d50_d40 = 0 mm, d101_d20 = 0 mm, d102_d21 = 30 deg, d114_d109 = 0 mm, d228_d227 = 0 mm, d229_d227 = 0 mm, d232_d227 = 0 mm, d233_d228_d227 = 0 mm, d234_d229_d227 = 0 mm, d235_d230 = 0 mm, d236_d231 = 0 mm, d248_d232_d227 = 0 mm, d249_d233_d228_d227 = 0 mm, d250_d234_d229_d227 = 0 mm, d251_d235_d230 = 0 mm, d252_d236_d231 = 0 mm, d262_d260 = 0 mm, d270_d269 = 0 mm
